# Autodesk Inventor assembly: tower1.2
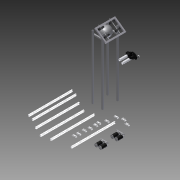
[picture p0: Inventor's stored thumbnail of the model, 180x180]
Saved by Autodesk Inventor 2011 SP1 (Build 150282100, 282)
## iProperties
Created: 2012-01-14
Part Number: tower1.2
Document SubType Name: Assembly
Designer: Christopher
Author: Christopher
## Documents named in this file (17)
- C:\Users\Christopher\Documents\Christopher\FIRST\Inventor files\2012\4 wheel kicker version 1\tower1.2.iam
- C:\Users\Christopher\Documents\Christopher\FIRST\Inventor files\2012\4 wheel kicker version 1\9 in .125 aluminum tube.ipt
- C:\Users\Christopher\Documents\Christopher\FIRST\Inventor files\2012\4 wheel kicker version 1\18 inch tube.ipt
- C:\Users\Christopher\Documents\Christopher\FIRST\Inventor files\2012\4 wheel kicker version 1\wheel.ipt
- C:\Users\Christopher\Documents\Christopher\FIRST\Inventor files\2012\4 wheel kicker version 1\axle1 .5inch.ipt
- C:\Users\Christopher\Documents\Christopher\FIRST\Inventor files\2012\tower first design\towerfrontdraft.ipt
- C:\Users\Christopher\Documents\Christopher\FIRST\Inventor files\2012\tower first design\towerbracebackwards.ipt
- C:\Users\Christopher\Documents\Christopher\FIRST\Inventor files\2012\tower first design\short thing.ipt
- C:\Users\Christopher\Documents\Christopher\FIRST\Inventor files\2012\tower first design\small axle.ipt
- C:\Users\Christopher\Documents\Christopher\FIRST\Inventor files\2012\tower first design\doorstop.ipt
- C:\Users\Christopher\Documents\Christopher\FIRST\Inventor files\2012\tower first design\towertallbackthing.ipt
- C:\Users\Christopher\Documents\Christopher\FIRST\Inventor files\2011\Kit of Parts\motors\Motors_FisherPrice_00968-9015.iam
- C:\Users\Christopher\Documents\Christopher\FIRST\Inventor files\2012\tower first design\pvc pipe 7inch.ipt
- C:\Users\Christopher\Documents\Christopher\FIRST\Inventor files\2011\Kit of Parts\Chassis\Chassis_Channel_AndyMark_am-0202.ipt
- C:\Users\Christopher\Documents\Christopher\FIRST\Inventor files\2011\Kit of Parts\Chassis\Chassis_CIMGearbox_AndyMark_am-0734.ipt
- C:\Users\Christopher\Documents\Christopher\FIRST\Inventor files\2011\Kit of Parts\Chassis\Chassis_CornerConnect_AndyMark_am-0212.ipt
- C:\Users\Christopher\Documents\Christopher\FIRST\Inventor files\2012\4 wheel kicker version 1\game ball.ipt
## Components (44 placed, 16 different names)
1. 18 inch tube:2 — Insert:1, Insert:2, Mate:1, Flush:1, Flush:2, Flush:3, Mate:6, Flush:12
2. wheel:1 — Insert:3
3. wheel:2 — Insert:4
4. wheel:3 — Insert:9
5. wheel:4 — Insert:10
6. axle1 .5inch:1 — Insert:1, Insert:3, Insert:9
7. axle1 .5inch:2 — Insert:2, Insert:4, Insert:10
8. 9 in .125 aluminum tube:1 — Mate:1, Flush:1, Flush:2, Mate:17, Flush:27, Flush:28, Insert:11, Insert:13
9. 9 in .125 aluminum tube:2 — Flush:3, Mate:6, Flush:12, Insert:12
10. towerfrontdraft:1 — Mate:10, Flush:19, Flush:20
11. towerfrontdraft:2 — Mate:9, Flush:17, Flush:18, Mate:18
12. towerbracebackwards:1 — Mate:10, Flush:19, Flush:20, Mate:15, Flush:26, Mate:22, Mate:23, Mate:24, Mate:26, Flush:31, Flush:32
13. towerbracebackwards:2 — Mate:9, Flush:17, Flush:18, Mate:13, Flush:25, Mate:19, Mate:20, Mate:21, Mate:25, Flush:29, Flush:30
14. short thing:1 — Mate:13, Flush:25, Insert:11, Mate:18
15. short thing:2 — Mate:15, Flush:26, Insert:12, Insert:14
16. 18 inch tube:3 — Mate:17, Flush:27, Flush:28
17. small axle:1 — Insert:13
18. small axle:2 — Insert:14
19. doorstop:1 — Mate:19, Mate:20, Mate:21
20. doorstop:2 — Mate:22, Mate:23, Mate:24
21. towertallbackthing:1 — Mate:26, Flush:31, Flush:32, Mate:27
22. towertallbackthing:2 — Mate:25, Flush:29, Flush:30
23. Motors_FisherPrice_00968-9015:2 [sub-assembly] — Mate:27, Insert:15, Insert:16
24. pvc pipe 7inch:1 — Insert:15, Insert:16
25. pvc pipe 7inch:2
26. Chassis_Channel_AndyMark_am-0202:1
27. Chassis_Channel_AndyMark_am-0202:2
28. Chassis_Channel_AndyMark_am-0202:3
29. Chassis_Channel_AndyMark_am-0202:4
30. Chassis_Channel_AndyMark_am-0202:5
31. Chassis_Channel_AndyMark_am-0202:6
32. Chassis_CIMGearbox_AndyMark_am-0734:1
33. Chassis_CIMGearbox_AndyMark_am-0734:2
34. Chassis_CornerConnect_AndyMark_am-0212:1
35. Chassis_CornerConnect_AndyMark_am-0212:2
36. Chassis_CornerConnect_AndyMark_am-0212:3
37. Chassis_CornerConnect_AndyMark_am-0212:4
38. Chassis_CornerConnect_AndyMark_am-0212:5
39. Chassis_CornerConnect_AndyMark_am-0212:6
40. Chassis_CornerConnect_AndyMark_am-0212:7
41. Chassis_CornerConnect_AndyMark_am-0212:8
42. Chassis_CornerConnect_AndyMark_am-0212:9
43. Chassis_CornerConnect_AndyMark_am-0212:10
44. game ball:1
## Relationships (45: Mate 17, Flush 16, Insert 12)
- Insert:1 (-12.7 mm): 18 inch tube:2 ↔ axle1 .5inch:1
- Insert:2 (-12.7 mm): 18 inch tube:2 ↔ axle1 .5inch:2
- Insert:3 (53.34 mm): wheel:1 ↔ axle1 .5inch:1
- Insert:4 (53.34 mm): wheel:2 ↔ axle1 .5inch:2
- Mate:1: 18 inch tube:2 ↔ 9 in .125 aluminum tube:1
- Flush:1: 18 inch tube:2 ↔ 9 in .125 aluminum tube:1
- Flush:2: 18 inch tube:2 ↔ 9 in .125 aluminum tube:1
- Insert:9 (193.04 mm): wheel:3 ↔ axle1 .5inch:1
- Insert:10 (193.04 mm): wheel:4 ↔ axle1 .5inch:2
- Flush:3: 18 inch tube:2 ↔ 9 in .125 aluminum tube:2
- Mate:6: 18 inch tube:2 ↔ 9 in .125 aluminum tube:2
- Flush:12: 18 inch tube:2 ↔ 9 in .125 aluminum tube:2
- Mate:9: towerfrontdraft:2 ↔ towerbracebackwards:2
- Flush:17: towerfrontdraft:2 ↔ towerbracebackwards:2
- Flush:18: towerfrontdraft:2 ↔ towerbracebackwards:2
- Mate:10: towerfrontdraft:1 ↔ towerbracebackwards:1
- Flush:19: towerfrontdraft:1 ↔ towerbracebackwards:1
- Flush:20: towerfrontdraft:1 ↔ towerbracebackwards:1
- Mate:13: towerbracebackwards:2 ↔ short thing:1
- Flush:25: towerbracebackwards:2 ↔ short thing:1
- Mate:15: towerbracebackwards:1 ↔ short thing:2
- Flush:26: towerbracebackwards:1 ↔ short thing:2
- Mate:17: 9 in .125 aluminum tube:1 ↔ 18 inch tube:3
- Flush:27: 9 in .125 aluminum tube:1 ↔ 18 inch tube:3
- Flush:28: 9 in .125 aluminum tube:1 ↔ 18 inch tube:3
- Insert:11 (15.875 mm): 9 in .125 aluminum tube:1 ↔ short thing:1
- Insert:12 (15.875 mm): 9 in .125 aluminum tube:2 ↔ short thing:2
- Insert:13 (-12.7 mm): 9 in .125 aluminum tube:1 ↔ small axle:1
- Insert:14 (-12.7 mm): short thing:2 ↔ small axle:2
- Mate:18 (-25.4 mm): towerfrontdraft:2 ↔ short thing:1
- Mate:19: towerbracebackwards:2 ↔ doorstop:1
- Mate:20 (-12.7 mm): towerbracebackwards:2 ↔ doorstop:1
- Mate:21 (-12.7 mm): towerbracebackwards:2 ↔ doorstop:1
- Mate:22: towerbracebackwards:1 ↔ doorstop:2
- Mate:23 (-12.7 mm): towerbracebackwards:1 ↔ doorstop:2
- Mate:24 (-12.7 mm): towerbracebackwards:1 ↔ doorstop:2
- Mate:25: towerbracebackwards:2 ↔ towertallbackthing:2
- Flush:29: towerbracebackwards:2 ↔ towertallbackthing:2
- Flush:30 (76.2 mm): towerbracebackwards:2 ↔ towertallbackthing:2
- Mate:26: towerbracebackwards:1 ↔ towertallbackthing:1
- Flush:31 (76.2 mm): towerbracebackwards:1 ↔ towertallbackthing:1
- Flush:32: towerbracebackwards:1 ↔ towertallbackthing:1
- Mate:27: towertallbackthing:1 ↔ Motors_FisherPrice_00968-9015:2
- Insert:15: Motors_FisherPrice_00968-9015:2 ↔ pvc pipe 7inch:1
- Insert:16: Motors_FisherPrice_00968-9015:2 ↔ pvc pipe 7inch:1
